# Autodesk Inventor assembly: 20mm Gantry Set
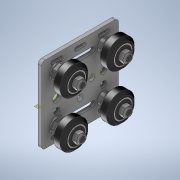
[picture p0: Inventor's stored thumbnail of the model, 180x180]
Saved by Autodesk Inventor 2020.3 (Build 243373000, 373)
## iProperties
Created: 2016-04-10
Part Number: 20mm Gantry Set
Document SubType Name: Assembly
Designer: Ben
Mass: 48.8675 g
Surface Area: 277.219 cm^2
Volume: 30.9657 cm^3
Density: 1.57812 g/cm^3
Author: Ben
## Documents named in this file (6)
- C:\Users\juanp\Desktop\ROBOCOL\Idea Final NAF\Gantry\Inventor\20mm Gantry Set.iam
- C:\Users\juanp\Desktop\ROBOCOL\Idea Final NAF\Gantry\Inventor\V-Slot Gantry Plate 20mm.ipt
- C:\Users\juanp\Desktop\ROBOCOL\Idea Final NAF\Gantry\Inventor\V-Wheel Solid Wheel.iam
- C:\Users\juanp\Desktop\ROBOCOL\Idea Final NAF\Gantry\Inventor\V-Wheel Solid Wheel - spacer.iam
- C:\Users\juanp\Desktop\ROBOCOL\Idea Final NAF\Gantry\Inventor\M5x25 low profile screw.ipt
- C:\Users\juanp\Desktop\ROBOCOL\Idea Final NAF\Gantry\Inventor\M5 Nylock.ipt
## Components (13 placed, 5 different names)
1. V-Slot Gantry Plate 20mm:1 — Mate:34, Mate:35, Mate:36, Mate:41, Mate:43, Mate:44, Mate:45, Mate:46, Mate:47, Mate:48, Mate:49, Angle:2, Angle:3, Angle:4, Mate:53, Mate:54, Mate:55
2. V-Wheel Solid Wheel:3 [sub-assembly] — Mate:12, Mate:26, Mate:48
3. V-Wheel Solid Wheel:4 [sub-assembly] — Mate:11, Mate:23, Mate:49
4. V-Wheel Solid Wheel - spacer:2 [sub-assembly] — Mate:24, Mate:41, Mate:42
5. M5x25 low profile screw:1 — Mate:11, Mate:19, Mate:45, Mate:47
6. M5x25 low profile screw:2 — Mate:12, Mate:20, Mate:46
7. M5x25 low profile screw:3 — Mate:22, Mate:43, Mate:44, Mate:42
8. M5 Nylock:1 — Mate:19, Mate:23, Angle:3
9. M5 Nylock:2 — Mate:20, Mate:26, Angle:4
10. M5 Nylock:4 — Mate:22, Mate:24, Angle:2
11. V-Wheel Solid Wheel - spacer:3 [sub-assembly] — Mate:54
12. M5x25 low profile screw:4 — Mate:53, Mate:55
13. M5 Nylock:5
## Relationships (30: Mate 26, Angle 3, Flush 1)
- Mate:11: V-Wheel Solid Wheel:4 ↔ M5x25 low profile screw:1
- Mate:12: V-Wheel Solid Wheel:3 ↔ M5x25 low profile screw:2
- Mate:19: M5x25 low profile screw:1 ↔ M5 Nylock:1
- Mate:20: M5x25 low profile screw:2 ↔ M5 Nylock:2
- Mate:22: M5x25 low profile screw:3 ↔ M5 Nylock:4
- Mate:23: V-Wheel Solid Wheel:4 ↔ M5 Nylock:1
- Mate:24: V-Wheel Solid Wheel - spacer:2 ↔ M5 Nylock:4
- Mate:26: V-Wheel Solid Wheel:3 ↔ M5 Nylock:2
- Flush:2
- Mate:34: V-Slot Gantry Plate 20mm:1
- Mate:35: V-Slot Gantry Plate 20mm:1
- Mate:36: V-Slot Gantry Plate 20mm:1
- Mate:41: V-Slot Gantry Plate 20mm:1 ↔ V-Wheel Solid Wheel - spacer:2
- Mate:42: V-Wheel Solid Wheel - spacer:2 ↔ M5x25 low profile screw:3
- Mate:43: V-Slot Gantry Plate 20mm:1 ↔ M5x25 low profile screw:3
- Mate:44: V-Slot Gantry Plate 20mm:1 ↔ M5x25 low profile screw:3
- Mate:45: V-Slot Gantry Plate 20mm:1 ↔ M5x25 low profile screw:1
- Mate:46: V-Slot Gantry Plate 20mm:1 ↔ M5x25 low profile screw:2
- Mate:47: V-Slot Gantry Plate 20mm:1 ↔ M5x25 low profile screw:1
- Mate:48: V-Slot Gantry Plate 20mm:1 ↔ V-Wheel Solid Wheel:3
- Mate:49: V-Slot Gantry Plate 20mm:1 ↔ V-Wheel Solid Wheel:4
- Angle:2 (0 deg): V-Slot Gantry Plate 20mm:1 ↔ M5 Nylock:4
- Angle:3 (0 deg): V-Slot Gantry Plate 20mm:1 ↔ M5 Nylock:1
- Angle:4 (0 deg): V-Slot Gantry Plate 20mm:1 ↔ M5 Nylock:2
- [Mate]: M5x25 low profile screw:4 ↔ M5 Nylock:5
- [Mate]: V-Wheel Solid Wheel - spacer:3 ↔ M5 Nylock:5
- [Mate]: V-Wheel Solid Wheel - spacer:3 ↔ M5x25 low profile screw:4
- Mate:53: V-Slot Gantry Plate 20mm:1 ↔ M5x25 low profile screw:4
- Mate:54: V-Slot Gantry Plate 20mm:1 ↔ V-Wheel Solid Wheel - spacer:3
- Mate:55: V-Slot Gantry Plate 20mm:1 ↔ M5x25 low profile screw:4
## Named parameters: d59_d21 = 0 mm, d60_d23 = 0 mm, d61_d47 = 0 mm
